# Autodesk Inventor assembly: EncoderV2.5
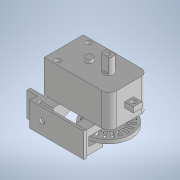
[picture p0: Inventor's stored thumbnail of the model, 180x180]
Saved by Autodesk Inventor 2022 (Build 260153070, 153G)
## iProperties
Created: 2022-01-31
Part Number: EncoderV2.5
Document SubType Name: Assembly
Designer: a laptop
Author: a laptop
## Documents named in this file (7)
- C:\Users\a laptop\Desktop\SumoBot\sumobotENCODER\EncoderV2\EncoderV2.5.iam
- C:\Users\a laptop\Desktop\SumoBot\sumobotENCODER\REF_PART\LM393 encoder.ipt
- C:\Users\a laptop\Desktop\SumoBot\sumobotENCODER\REF_PART\TT encoder disk.ipt
- C:\Users\a laptop\Desktop\SumoBot\sumobotENCODER\REF_PART\TT motor output.ipt
- C:\Users\a laptop\Desktop\SumoBot\sumobotENCODER\REF_PART\TTencoderspacer.ipt
- C:\Users\a laptop\Desktop\SumoBot\sumobotENCODER\EncoderV2\EncoderV2CAP.ipt
- C:\Users\a laptop\Desktop\SumoBot\sumobotENCODER\EncoderV2\ENCODERV2PLATE.ipt
## Components (6 placed, 6 different names)
1. LM393 encoder:1 — Mate:8, Mate:12
2. TT encoder disk:1 — Mate:3, Mate:4, Mate:5, Mate:6
3. TT motor output:1 — Mate:1, Mate:2, Mate:4, Mate:5, Mate:7, Mate:9, Mate:10, Mate:11
4. TTencoderspacer:1 — Mate:1, Mate:2, Mate:3
5. EncoderV2CAP:1 — Mate:6, Mate:7
6. ENCODERV2PLATE:1 — Mate:8, Mate:9, Mate:10, Mate:11, Mate:12
## Relationships (12: Mate 12)
- Mate:1: TT motor output:1 ↔ TTencoderspacer:1
- Mate:2: TT motor output:1 ↔ TTencoderspacer:1
- Mate:3: TT encoder disk:1 ↔ TTencoderspacer:1
- Mate:4: TT encoder disk:1 ↔ TT motor output:1
- Mate:5: TT encoder disk:1 ↔ TT motor output:1
- Mate:6: TT encoder disk:1 ↔ EncoderV2CAP:1
- Mate:7: TT motor output:1 ↔ EncoderV2CAP:1
- Mate:8: LM393 encoder:1 ↔ ENCODERV2PLATE:1
- Mate:9: TT motor output:1 ↔ ENCODERV2PLATE:1
- Mate:10: TT motor output:1 ↔ ENCODERV2PLATE:1
- Mate:11: TT motor output:1 ↔ ENCODERV2PLATE:1
- Mate:12: LM393 encoder:1 ↔ ENCODERV2PLATE:1
